# Autodesk Inventor assembly: Assembly in
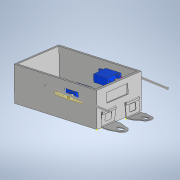
[picture p0: Inventor's stored thumbnail of the model, 180x180]
Saved by Autodesk Inventor 2021 (Build 250183000, 183)
## iProperties
Created: 2021-07-06
Part Number: Assembly in
Document SubType Name: Assembly
Designer: Sahana
Author: Sahana
## Documents named in this file (7)
- E:\project 1\EE\Assembly in.iam
- E:\project 1\EE\rectangular box.ipt
- E:\project 1\EE\Servo Motor SG90.ipt
- E:\project 1\EE\horn.ipt
- E:\project 1\EE\Bolt.ipt
- E:\project 1\EE\cane stick (1).ipt
- E:\project 1\sheet metal part\sheet metal part.ipt
## Components (13 placed, 6 different names)
1. rectangular box:1 — Mate:1, Mate:2, Mate:4, Mate:10, Mate:11
2. Servo Motor SG90:1 — Mate:1, Mate:3, Mate:5, Mate:8
3. Servo Motor SG90:2 — Mate:2, Mate:6, Mate:7, Mate:9
4. Bolt:1 — Mate:6
5. Bolt:2 — Mate:7
6. Bolt:3 — Mate:5
7. Bolt:4 — Mate:3, Mate:4
8. cane stick (1):1 — Mate:12
9. cane stick (1):2 — Mate:13
10. horn:1 — Mate:8, Mate:12
11. horn:2 — Mate:9, Mate:13
12. sheet metal part:1 — Mate:11
13. sheet metal part:2 — Mate:10
## Relationships (13: Mate 13)
- Mate:1: rectangular box:1 ↔ Servo Motor SG90:1
- Mate:2: rectangular box:1 ↔ Servo Motor SG90:2
- Mate:3: Servo Motor SG90:1 ↔ Bolt:4
- Mate:4: rectangular box:1 ↔ Bolt:4
- Mate:5: Servo Motor SG90:1 ↔ Bolt:3
- Mate:6: Servo Motor SG90:2 ↔ Bolt:1
- Mate:7: Servo Motor SG90:2 ↔ Bolt:2
- Mate:8: Servo Motor SG90:1 ↔ horn:1
- Mate:9: Servo Motor SG90:2 ↔ horn:2
- Mate:10: rectangular box:1 ↔ sheet metal part:2
- Mate:11: rectangular box:1 ↔ sheet metal part:1
- Mate:12: cane stick (1):1 ↔ horn:1
- Mate:13: cane stick (1):2 ↔ horn:2
